# Autodesk Inventor assembly: Polycarb main conv
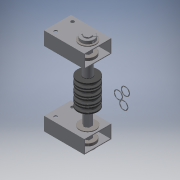
[picture p0: Inventor's stored thumbnail of the model, 180x180]
Saved by Autodesk Inventor 2018 (Build 220112000, 112)
## iProperties
Created: 2020-01-27
Part Number: Polycarb main conv
Document SubType Name: Assembly
Designer: Burni
Author: Burni
## Documents named in this file (8)
- H:\GitHub\2020CAD\Tyler's Ball Storage\Polycarb main conv.iam
- H:\GitHub\2020CAD\Tyler's Ball Storage\Hex shaft\Shooter hex shaft.ipt
- H:\GitHub\2020CAD\Tyler's Ball Storage\1x2 hexshaft mount.ipt
- H:\GitHub\2020CAD\Tyler's Ball Storage\am-2986 FR8ZZ Hex Bearing.ipt
- H:\GitHub\2020CAD\Tyler's Ball Storage\WCP-0096 Rev1.ipt
- H:\GitHub\2020CAD\Tyler's Ball Storage\Other parts\Clamping_Shaft_Collar_-_1_2_Hex_ID_217-2737.ipt
- H:\GitHub\2020CAD\Tyler's Ball Storage\Spacers\.021''spacer.ipt
- H:\GitHub\2020CAD\Tyler's Ball Storage\Spacers\1.59''spacer.ipt
## Components (17 placed, 7 different names)
1. Shooter hex shaft:1 — Mate:10, Mate:11, Mate:12, Mate:13, Mate:14, Mate:15, Mate:16, Mate:17, Mate:19, Mate:20, Flush:6, Mate:23, Mate:25, Mate:27, Mate:28, Mate:30, Mate:31, Mate:34, Mate:35
2. 1x2 hexshaft mount:1 — Mate:1, Mate:2, Mate:3, Mate:5, Flush:4, Flush:5, Mate:21, Mate:22
3. 1x2 hexshaft mount:2 — Mate:6, Mate:7, Mate:8, Mate:9, Flush:4, Flush:5, Mate:21, Flush:6
4. am-2986 FR8ZZ Hex Bearing:1 — Mate:7, Mate:8, Mate:12, Mate:13
5. am-2986 FR8ZZ Hex Bearing:2 — Mate:6, Mate:9, Mate:10, Mate:11, Mate:32
6. am-2986 FR8ZZ Hex Bearing:3 — Mate:1, Mate:2, Flush:2, Mate:14, Mate:15, Mate:33
7. am-2986 FR8ZZ Hex Bearing:4 — Mate:3, Mate:5, Flush:2, Mate:29
8. WCP-0096 Rev1:2 — Mate:16, Mate:17, Mate:18, Mate:22
9. WCP-0096 Rev1:3 — Mate:18, Mate:19, Mate:20, Mate:24
10. WCP-0096 Rev1:4 — Mate:23, Mate:24, Mate:26
11. WCP-0096 Rev1:5 — Mate:25, Mate:26
12. Clamping_Shaft_Collar_-_1_2_Hex_ID_217-2737:1 — Mate:27, Mate:28, Mate:29
13. Clamping_Shaft_Collar_-_1_2_Hex_ID_217-2737:2 — Mate:30, Mate:31, Mate:32
14. .021''spacer:1
15. .021''spacer:2
16. .021''spacer:3
17. 1.59''spacer:1 — Mate:33, Mate:34, Mate:35
## Relationships (38: Mate 34, Flush 4)
- Mate:1: 1x2 hexshaft mount:1 ↔ am-2986 FR8ZZ Hex Bearing:3
- Mate:2: 1x2 hexshaft mount:1 ↔ am-2986 FR8ZZ Hex Bearing:3
- Mate:3: 1x2 hexshaft mount:1 ↔ am-2986 FR8ZZ Hex Bearing:4
- Mate:5: 1x2 hexshaft mount:1 ↔ am-2986 FR8ZZ Hex Bearing:4
- Mate:6: 1x2 hexshaft mount:2 ↔ am-2986 FR8ZZ Hex Bearing:2
- Mate:7: 1x2 hexshaft mount:2 ↔ am-2986 FR8ZZ Hex Bearing:1
- Mate:8: 1x2 hexshaft mount:2 ↔ am-2986 FR8ZZ Hex Bearing:1
- Mate:9: 1x2 hexshaft mount:2 ↔ am-2986 FR8ZZ Hex Bearing:2
- Mate:10: Shooter hex shaft:1 ↔ am-2986 FR8ZZ Hex Bearing:2
- Mate:11: Shooter hex shaft:1 ↔ am-2986 FR8ZZ Hex Bearing:2
- Mate:12: Shooter hex shaft:1 ↔ am-2986 FR8ZZ Hex Bearing:1
- Mate:13: Shooter hex shaft:1 ↔ am-2986 FR8ZZ Hex Bearing:1
- Flush:2: am-2986 FR8ZZ Hex Bearing:3 ↔ am-2986 FR8ZZ Hex Bearing:4
- Mate:14: Shooter hex shaft:1 ↔ am-2986 FR8ZZ Hex Bearing:3
- Mate:15: Shooter hex shaft:1 ↔ am-2986 FR8ZZ Hex Bearing:3
- Flush:4: 1x2 hexshaft mount:1 ↔ 1x2 hexshaft mount:2
- Flush:5: 1x2 hexshaft mount:1 ↔ 1x2 hexshaft mount:2
- Mate:16: Shooter hex shaft:1 ↔ WCP-0096 Rev1:2
- Mate:17: Shooter hex shaft:1 ↔ WCP-0096 Rev1:2
- Mate:18 (28.575 mm): WCP-0096 Rev1:2 ↔ WCP-0096 Rev1:3
- Mate:19: Shooter hex shaft:1 ↔ WCP-0096 Rev1:3
- Mate:20: Shooter hex shaft:1 ↔ WCP-0096 Rev1:3
- Mate:21 (114.3 mm): 1x2 hexshaft mount:1 ↔ 1x2 hexshaft mount:2
- Flush:6 (9.525 mm): Shooter hex shaft:1 ↔ 1x2 hexshaft mount:2
- Mate:22 (31.75 mm): 1x2 hexshaft mount:1 ↔ WCP-0096 Rev1:2
- Mate:23: Shooter hex shaft:1 ↔ WCP-0096 Rev1:4
- Mate:24 (0.5292 mm): WCP-0096 Rev1:3 ↔ WCP-0096 Rev1:4
- Mate:25: Shooter hex shaft:1 ↔ WCP-0096 Rev1:5
- Mate:26 (0.5292 mm): WCP-0096 Rev1:4 ↔ WCP-0096 Rev1:5
- Mate:27: Shooter hex shaft:1 ↔ Clamping_Shaft_Collar_-_1_2_Hex_ID_217-2737:1
- Mate:28: Shooter hex shaft:1 ↔ Clamping_Shaft_Collar_-_1_2_Hex_ID_217-2737:1
- Mate:29: am-2986 FR8ZZ Hex Bearing:4 ↔ Clamping_Shaft_Collar_-_1_2_Hex_ID_217-2737:1
- Mate:30: Shooter hex shaft:1 ↔ Clamping_Shaft_Collar_-_1_2_Hex_ID_217-2737:2
- Mate:31: Shooter hex shaft:1 ↔ Clamping_Shaft_Collar_-_1_2_Hex_ID_217-2737:2
- Mate:32: am-2986 FR8ZZ Hex Bearing:2 ↔ Clamping_Shaft_Collar_-_1_2_Hex_ID_217-2737:2
- Mate:33: am-2986 FR8ZZ Hex Bearing:3 ↔ 1.59''spacer:1
- Mate:34: Shooter hex shaft:1 ↔ 1.59''spacer:1
- Mate:35: Shooter hex shaft:1 ↔ 1.59''spacer:1
